# Autodesk Inventor assembly: EnsamblajeLevitador
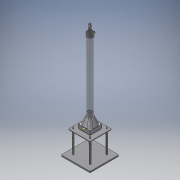
[picture p0: Inventor's stored thumbnail of the model, 180x180]
Saved by Autodesk Inventor 2017 (Build 210142000, 142)
## iProperties
Part Number: EnsamblajeLevitador
Material: Genérico
Document SubType Name: Assembly
Designer: Leonardo
Author: Leonardo
## Documents named in this file (10)
- C:\Users\Leonardo\Documents\Universidad\02 Control\Control Edgar\Laboratorio\02 Cad\EnsamblajeLevitador.iam
- C:\Users\Leonardo\Documents\Universidad\02 Control\Control Edgar\Laboratorio\02 Cad\fan80mmx20mm.iam
- C:\Users\Leonardo\Documents\Universidad\02 Control\Control Edgar\Laboratorio\02 Cad\Tubo33mmx50cm.ipt
- C:\Users\Leonardo\Documents\Universidad\02 Control\Control Edgar\Laboratorio\02 Cad\TolvaReductora.ipt
- C:\Users\Leonardo\Documents\Universidad\02 Control\Control Edgar\Laboratorio\02 Cad\TablaSoporte1.ipt
- C:\Users\Leonardo\Documents\Universidad\02 Control\Control Edgar\Laboratorio\02 Cad\TablaSoporte2.ipt
- C:\Users\Leonardo\Documents\Universidad\02 Control\Control Edgar\Laboratorio\02 Cad\TrnlloSinFin.ipt
- C:\Users\Leonardo\Documents\Universidad\02 Control\Control Edgar\Laboratorio\02 Cad\Resorte.ipt
- C:\Users\Leonardo\Documents\Universidad\02 Control\Control Edgar\Laboratorio\02 Cad\SoporteSensor.ipt
- C:\Users\Leonardo\Documents\Universidad\02 Control\Control Edgar\Laboratorio\02 Cad\SensorCJMCU530.ipt
## Components (12 placed, 9 different names)
1. fan80mmx20mm:1 [sub-assembly] — Coincidencia:1, Coincidencia:2, Nivelación:1, Nivelación:2
2. Tubo33mmx50cm:1 — Coincidencia:1, Coincidencia:2, Coincidencia:3, Coincidencia:4
3. TolvaReductora:1 — Nivelación:1
4. TablaSoporte1:1 — Nivelación:2, Nivelación:3, Nivelación:4
5. TablaSoporte2:1 — Nivelación:3, Nivelación:4, Nivelación:5
6. TrnlloSinFin:1 — Nivelación:5
7. Resorte:1
8. Resorte:2
9. Resorte:3
10. Resorte:4
11. SoporteSensor:1 — Coincidencia:3, Coincidencia:4, Nivelación:6
12. SensorCJMCU530:1 — Nivelación:6
## Relationships (10: Flush 6, Mate 4)
- Coincidencia:1 [Mate]: fan80mmx20mm:1 ↔ Tubo33mmx50cm:1
- Coincidencia:2 [Mate] (55.5 mm): fan80mmx20mm:1 ↔ Tubo33mmx50cm:1
- Nivelación:1 [Flush]: fan80mmx20mm:1 ↔ TolvaReductora:1
- Nivelación:2 [Flush]: fan80mmx20mm:1 ↔ TablaSoporte1:1
- Nivelación:3 [Flush]: TablaSoporte1:1 ↔ TablaSoporte2:1
- Nivelación:4 [Flush] (150 mm): TablaSoporte1:1 ↔ TablaSoporte2:1
- Nivelación:5 [Flush]: TablaSoporte2:1 ↔ TrnlloSinFin:1
- Coincidencia:3 [Mate]: Tubo33mmx50cm:1 ↔ SoporteSensor:1
- Coincidencia:4 [Mate]: Tubo33mmx50cm:1 ↔ SoporteSensor:1
- Nivelación:6 [Flush]: SoporteSensor:1 ↔ SensorCJMCU530:1
